# Autodesk Inventor assembly: Assembly - Load Cell
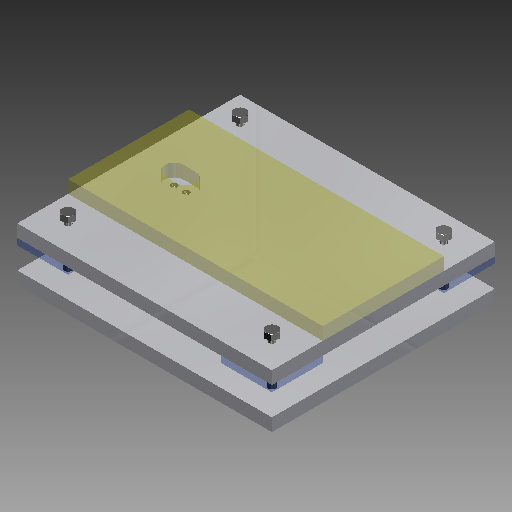
[picture p0: Inventor's stored thumbnail of the model, 512x512]
Saved by Autodesk Inventor 2018.1 (Build 221171000, 171)
## iProperties
Created: 2017-07-26
Part Number: Assembly - Load Cell
Document SubType Name: Assembly
Designer: Tom
Author: Tom
## Documents named in this file (9)
- \\Mac\Dropbox\2015-2016\Bachelorproef\Inventor\Etstank_v2\load cell_assembly.iam
- \\Mac\Dropbox\2015-2016\Bachelorproef\Inventor\Etstank_v2\load cell.ipt
- \\Mac\Dropbox\2015-2016\Bachelorproef\Inventor\Etstank_v2\platform_top.ipt
- \\Mac\Dropbox\2015-2016\Bachelorproef\Inventor\Etstank_v2\platform_bottom.ipt
- \\Mac\Dropbox\2015-2016\Bachelorproef\Inventor\Etstank_v2\load cell_spacer.ipt
- \\Mac\Dropbox\2015-2016\Bachelorproef\Inventor\Etstank_v2\platform_nut_holder_assembly.iam
- \\Mac\Dropbox\2015-2016\Bachelorproef\Inventor\Etstank_v2\pltaform_support plate.ipt
- \\Mac\Home\Documents\Inventor\Content Center Files\R2018\en-US\ANSI B18.3.1M(2)\ANSI B18.3.1M - M6x1 x 20(6).ipt
- \\Mac\Dropbox\2015-2016\Bachelorproef\Inventor\Etstank_v2\par.xls
## Components (14 placed, 7 different names)
1. load cell:1 — Flush:1, Flush:2, Mate:3, Mate:4, Mate:7, Mate:8, Mate:9, Mate:10, Mate:11, Mate:12
2. platform_top:1 — Flush:1, Flush:2, Flush:3, Flush:4, Flush:5, Flush:6, Mate:14
3. platform_bottom:1 — Flush:3, Flush:4, Flush:7, Flush:8, Mate:13, Flush:9, Flush:10, Mate:17, Flush:11, Flush:12, Flush:13, Flush:14, Flush:15, Flush:16, Mate:18, Mate:19, Mate:20, Mate:21, Flush:17, Flush:18, Mate:22, Mate:23
4. Drilled Broached Hexagon Socket Head Cap Screw - 2 Holes - Metric M6x1 x 20:5 — Flush:8, Mate:22
5. Drilled Broached Hexagon Socket Head Cap Screw - 2 Holes - Metric M6x1 x 20:6 — Flush:7, Mate:23
6. Drilled Broached Hexagon Socket Head Cap Screw - 2 Holes - Metric M6x1 x 20:7 — Mate:4, Flush:6
7. Drilled Broached Hexagon Socket Head Cap Screw - 2 Holes - Metric M6x1 x 20:8 — Mate:3, Flush:5
8. load cell_spacer:1 — Mate:7, Mate:9, Mate:10, Mate:14
9. load cell_spacer:2 — Mate:8, Mate:11, Mate:12, Mate:13
10. platform_nut_holder_assembly:1 [sub-assembly] — Flush:9, Flush:10, Mate:17
11. platform_nut_holder_assembly:2 [sub-assembly] — Flush:12, Flush:13, Mate:20
12. platform_nut_holder_assembly:3 [sub-assembly] — Flush:11, Flush:14, Mate:19
13. platform_nut_holder_assembly:4 [sub-assembly] — Flush:15, Flush:16, Mate:18
14. pltaform_support plate:1 — Mate:21, Flush:17, Flush:18
## Relationships (35: Flush 18, Mate 17)
- Flush:1 (165 mm): load cell:1 ↔ platform_top:1
- Flush:2 (184.525 mm): load cell:1 ↔ platform_top:1
- Flush:3: platform_top:1 ↔ platform_bottom:1
- Flush:4: platform_top:1 ↔ platform_bottom:1
- Mate:3: load cell:1 ↔ Drilled Broached Hexagon Socket Head Cap Screw - 2 Holes - Metric M6x1 x 20:8
- Mate:4: load cell:1 ↔ Drilled Broached Hexagon Socket Head Cap Screw - 2 Holes - Metric M6x1 x 20:7
- Flush:5: platform_top:1 ↔ Drilled Broached Hexagon Socket Head Cap Screw - 2 Holes - Metric M6x1 x 20:8
- Flush:6: platform_top:1 ↔ Drilled Broached Hexagon Socket Head Cap Screw - 2 Holes - Metric M6x1 x 20:7
- Flush:7: platform_bottom:1 ↔ Drilled Broached Hexagon Socket Head Cap Screw - 2 Holes - Metric M6x1 x 20:6
- Flush:8: platform_bottom:1 ↔ Drilled Broached Hexagon Socket Head Cap Screw - 2 Holes - Metric M6x1 x 20:5
- Mate:7: load cell:1 ↔ load cell_spacer:1
- Mate:8: load cell:1 ↔ load cell_spacer:2
- Mate:9: load cell:1 ↔ load cell_spacer:1
- Mate:10: load cell:1 ↔ load cell_spacer:1
- Mate:11: load cell:1 ↔ load cell_spacer:2
- Mate:12: load cell:1 ↔ load cell_spacer:2
- Mate:13: platform_bottom:1 ↔ load cell_spacer:2
- Mate:14: platform_top:1 ↔ load cell_spacer:1
- Flush:9: platform_bottom:1 ↔ platform_nut_holder_assembly:1
- Flush:10: platform_bottom:1 ↔ platform_nut_holder_assembly:1
- Mate:17: platform_bottom:1 ↔ platform_nut_holder_assembly:1
- Flush:11: platform_bottom:1 ↔ platform_nut_holder_assembly:3
- Flush:12: platform_bottom:1 ↔ platform_nut_holder_assembly:2
- Flush:13: platform_bottom:1 ↔ platform_nut_holder_assembly:2
- Flush:14: platform_bottom:1 ↔ platform_nut_holder_assembly:3
- Flush:15: platform_bottom:1 ↔ platform_nut_holder_assembly:4
- Flush:16: platform_bottom:1 ↔ platform_nut_holder_assembly:4
- Mate:18: platform_bottom:1 ↔ platform_nut_holder_assembly:4
- Mate:19: platform_bottom:1 ↔ platform_nut_holder_assembly:3
- Mate:20: platform_bottom:1 ↔ platform_nut_holder_assembly:2
- Mate:21: platform_bottom:1 ↔ pltaform_support plate:1
- Flush:17 (80 mm): platform_bottom:1 ↔ pltaform_support plate:1
- Flush:18: platform_bottom:1 ↔ pltaform_support plate:1
- Mate:22: platform_bottom:1 ↔ Drilled Broached Hexagon Socket Head Cap Screw - 2 Holes - Metric M6x1 x 20:5
- Mate:23: platform_bottom:1 ↔ Drilled Broached Hexagon Socket Head Cap Screw - 2 Holes - Metric M6x1 x 20:6
## Named parameters: maxh = 400 mm, maxw = 350 mm, lcsd = 19.05 mm, lcdd = 100 mm, lcwd1 = 25 mm, lcwd2 = 34 mm, lcw = 20 mm, lch1 = 39 mm, lch2 = 40 mm, lcl = 150 mm, lcwd3 = 43 mm, dia1 = 6 mm, td = 18 mm, bhh = 6 mm, bhd = 10 mm, sw = 25 mm, sh = 31 mm, spacert = 2 mm, nutdist = 40 mm, platft = 20 mm, supt = 20 mm, pvct = 5 mm, dia4 = 11 mm, actual_tankv = 1.4023e+07 mm, dia2 = 20 mm, tankv = 1e+07 mm, dia3 = 8 mm, tankl = 379 mm, tankw = 100 mm, tankh = 370 mm, play = 9 mm, holeh = 26 mm, surroundh = 60 mm, slack = 0.5 mm, surroundt = 5 mm, play2 = 3 mm, maxl = 400 mm, diaoverflow = 25 mm, extra_height = 100 mm, diaph = 32 mm, diacucl = 32 mm, diawater = 25 mm, diaair = 32 mm, mindist = 80 mm, distfromedge = 10 mm, diasurroundhole = 42 mm, sensorsupportl = 100 mm, brachetw = 10 mm, diagrate = 12 mm, gratespacing = 12.02082 mm, sidedist = 13.9375 mm, bottomdist = 9.6355 mm, diafloat = 50 mm, diahcl = 32 mm, bracketw = 10 mm, bracketwtop = 6 mm, bracketwbottom = 6 mm, handlesupporth = 20 mm, handlew = 50 mm, handlel = 120 mm, nett = 1 mm, nethole = 16 mm, nettop = 7 mm, netside = 3.5 mm, netholespacing = 2 mm, nutholdert = 10 mm, diaetape = 32 mm
